# Autodesk Inventor assembly: QRE MiniBoards 1
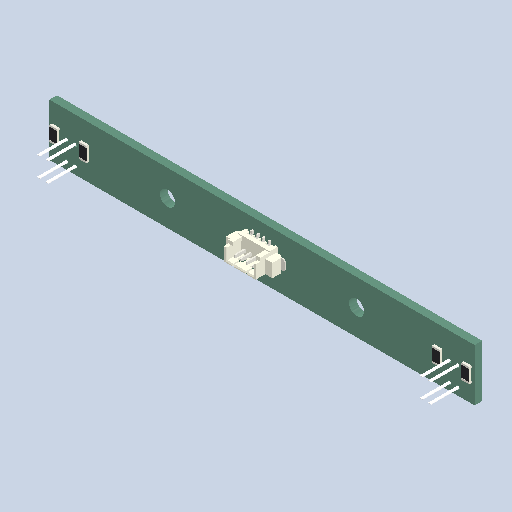
[picture p0: Inventor's stored thumbnail of the model, 512x512]
Saved by Autodesk Inventor 2024 (Build 280153000, 153)
## iProperties
Company: Kicad
Created: 2024-01-26
Part Number: QRE MiniBoards 1
Description: KiCad electronic assembly
Document SubType Name: Assembly
Designer: jaryj
Authority: Unknown
Sending System: KiCad to STEP converter
Preprocessor: Open CASCADE STEP processor 7.6
Title: QRE MiniBoards.step
Author: Pcbnew
## Documents named in this file (5)
- C:\Users\Simak\OneDrive\Dokumenty\GitHub\RoboCop\- 3D -\PCBs\QRE MiniBoards\QRE MiniBoards\QRE MiniBoards.iam
- C:\Users\Simak\OneDrive\Dokumenty\GitHub\RoboCop\- 3D -\PCBs\QRE MiniBoards\QRE MiniBoards\R_1206_3216Metric.iam
- C:\Users\Simak\OneDrive\Dokumenty\GitHub\RoboCop\- 3D -\PCBs\QRE MiniBoards\QRE MiniBoards\Molex_PicoBlade_53398-0471_1x04-1MP_P1.25mm_Vertical.iam
- C:\Users\Simak\OneDrive\Dokumenty\GitHub\RoboCop\- 3D -\PCBs\QRE MiniBoards\QRE MiniBoards\QRE1113.iam
- C:\Users\Simak\OneDrive\Dokumenty\GitHub\RoboCop\- 3D -\PCBs\QRE MiniBoards\QRE MiniBoards\QRE MiniBoards PCB.ipt
## Components (8 placed, 8 different names)
1. 2 [sub-assembly]
2. 4 [sub-assembly]
3. 5 [sub-assembly]
4. 6 [sub-assembly]
5. 7 [sub-assembly]
6. 9 [sub-assembly] — Stejný směr:1
7. 10 [sub-assembly] — Stejný směr:1
8. 11
## Relationships (1: Flush 1)
- Stejný směr:1 [Flush]: 9 ↔ 10
